# Autodesk Inventor assembly: Car
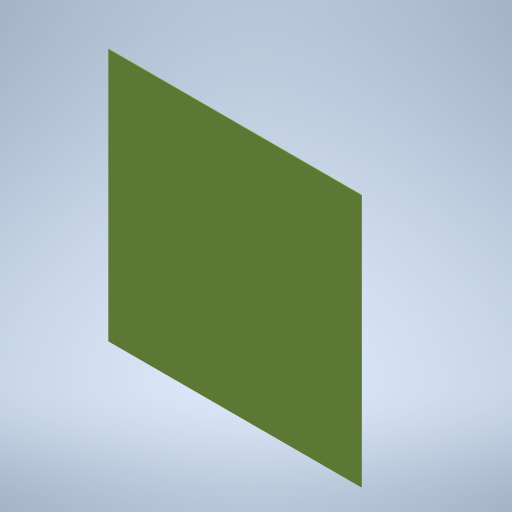
[picture p0: Inventor's stored thumbnail of the model, 512x512]
Saved by Autodesk Inventor 2024 (Build 280153000, 153)
## iProperties
Created: 2022-11-29
Part Number: Car
Document SubType Name: Assembly
Designer: kakik
Author: kakik
## Documents named in this file (11)
- C:\Users\kakik\OneDrive\Desktop\football-car-computer-vision\Dev\CAD_Files\Car.iam
- C:\Users\kakik\OneDrive\Desktop\football-car-computer-vision\Dev\CAD_Files\Base.ipt
- C:\Users\kakik\OneDrive\Desktop\football-car-computer-vision\Dev\CAD_Files\motor.ipt
- C:\Users\kakik\OneDrive\Desktop\football-car-computer-vision\Dev\CAD_Files\Tyre\Tyre.iam
- C:\Users\kakik\OneDrive\Desktop\football-car-computer-vision\Dev\CAD_Files\grass.ipt
- C:\Users\kakik\OneDrive\Desktop\football-car-computer-vision\Dev\CAD_Files\rearaxle.ipt
- C:\Users\kakik\OneDrive\Desktop\football-car-computer-vision\Dev\CAD_Files\Norm\M3_F_TO_F_10MM_STANDOFF.ipt
- C:\Users\kakik\OneDrive\Desktop\football-car-computer-vision\Dev\CAD_Files\sidemotor.ipt
- C:\Users\kakik\OneDrive\Desktop\football-car-computer-vision\Dev\CAD_Files\Claw\Claw5.ipt
- C:\Users\kakik\OneDrive\Desktop\p2\Ball\Ball.iam
- C:\Users\kakik\OneDrive\Desktop\p2\Claw\Claw3.ipt
## Components (14 placed, 10 different names)
1. Base:1 — Mate:1, Flush:1, Mate:2, Mate:3, Flush:3, Mate:5, Mate:6, Mate:15, Mate:16, Mate:17, Mate:18, Mate:27, Mate:37, Flush:8, Mate:38, Mate:43, Mate:47, Mate:49, Mate:50, Mate:51, Mate:52, Mate:53
2. motor:1 — Mate:1, Flush:1, Mate:2, Flush:2
3. motor:2 — Mate:3, Flush:2, Flush:3, Mate:4
4. Tyre:1 [sub-assembly] — Mate:4, Mate:5, Mate:7, Tangent:2
5. Tyre:2 [sub-assembly] — Mate:6, Mate:7
6. grass:1 — Tangent:1, Tangent:2, Mate:18, Mate:45
7. rearaxle:1 — Mate:15, Mate:16, Mate:17, Tangent:1
8. M3_F_TO_F_10MM_STANDOFF:1 — Mate:27, Mate:46, Mate:49
9. M3_F_TO_F_10MM_STANDOFF:2 — Mate:47, Mate:48
10. sidemotor:1 — Mate:37, Flush:8, Flush:9, Flush:10, Mate:50
11. sidemotor:2 — Mate:38, Flush:9, Flush:10
12. Claw5:1 — Mate:43, Mate:46, Mate:48, Mate:51, Flush:11
13. Claw3:1 — Mate:52, Mate:53, Flush:11
14. Ball:1 [sub-assembly] — Mate:45
## Relationships (33: Mate 24, Flush 7, Tangent 2)
- Mate:1: Base:1 ↔ motor:1
- Flush:1 (3 mm): Base:1 ↔ motor:1
- Mate:2: Base:1 ↔ motor:1
- Mate:3: Base:1 ↔ motor:2
- Flush:2: motor:1 ↔ motor:2
- Flush:3 (3 mm): Base:1 ↔ motor:2
- Mate:4: motor:2 ↔ Tyre:1
- Mate:5 (2 mm): Base:1 ↔ Tyre:1
- Mate:6 (2 mm): Base:1 ↔ Tyre:2
- Mate:7: Tyre:1 ↔ Tyre:2
- Mate:15 (10 mm): Base:1 ↔ rearaxle:1
- Mate:16: Base:1 ↔ rearaxle:1
- Mate:17: Base:1 ↔ rearaxle:1
- Tangent:1: grass:1 ↔ rearaxle:1
- Tangent:2: Tyre:1 ↔ grass:1
- Mate:18: Base:1 ↔ grass:1
- Mate:27: Base:1 ↔ M3_F_TO_F_10MM_STANDOFF:1
- Mate:37: Base:1 ↔ sidemotor:1
- Flush:8 (-10 mm): Base:1 ↔ sidemotor:1
- Mate:38: Base:1 ↔ sidemotor:2
- Flush:9: sidemotor:1 ↔ sidemotor:2
- Flush:10: sidemotor:1 ↔ sidemotor:2
- Mate:43: Base:1 ↔ Claw5:1
- Mate:45 (30 mm): grass:1 ↔ Ball:1
- Mate:46: M3_F_TO_F_10MM_STANDOFF:1 ↔ Claw5:1
- Mate:47: Base:1 ↔ M3_F_TO_F_10MM_STANDOFF:2
- Mate:48: M3_F_TO_F_10MM_STANDOFF:2 ↔ Claw5:1
- Mate:49: Base:1 ↔ M3_F_TO_F_10MM_STANDOFF:1
- Mate:50: Base:1 ↔ sidemotor:1
- Mate:51: Base:1 ↔ Claw5:1
- Mate:52: Base:1 ↔ Claw3:1
- Mate:53: Base:1 ↔ Claw3:1
- Flush:11: Claw5:1 ↔ Claw3:1
